# Autodesk Inventor assembly: Nose assembly
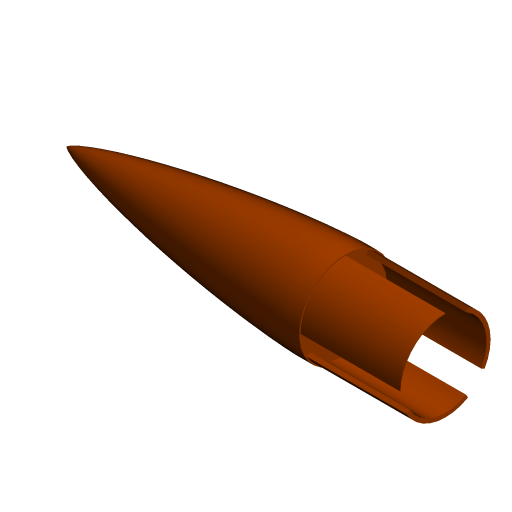
[picture p0: Inventor's stored thumbnail of the model, 512x512]
Saved by Autodesk Inventor 2024 (Build 280153000, 153)
## iProperties
Part Number: Nose assembly
Document SubType Name: Assembly
Designer: Jamie
Author: Jamie
## Documents named in this file (3)
- C:\Users\Jamie\Documents\Uni\DARE\Scrambler-2-CAD\Autodesk\Nose assembly.iam
- C:\Users\Jamie\Documents\Uni\DARE\Scrambler-2-CAD\Autodesk\smoke_grenade.ipt
- C:\Users\Jamie\Documents\Uni\DARE\Scrambler-2-CAD\Autodesk\Nosecone.ipt
## Components (2 placed, 2 different names)
1. smoke_grenade:1 — Mate:1, Mate:2
2. Nosecone:1 — Mate:1, Mate:2
## Relationships (2: Mate 2)
- Mate:1: smoke_grenade:1 ↔ Nosecone:1
- Mate:2: smoke_grenade:1 ↔ Nosecone:1
